# Autodesk Inventor assembly: Case inferiore completo
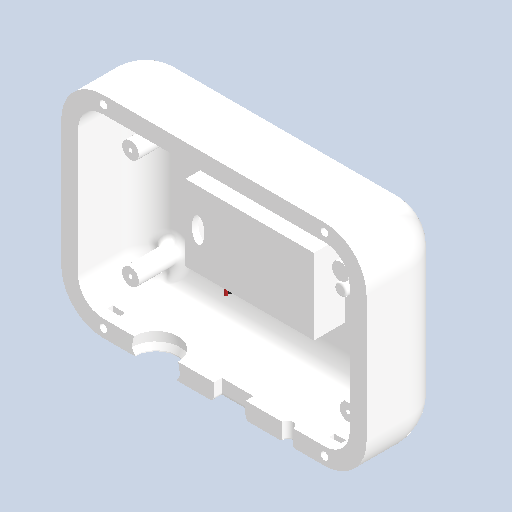
[picture p0: Inventor's stored thumbnail of the model, 512x512]
Saved by Autodesk Inventor 2023 (Build 270158000, 158)
## iProperties
Created: 2022-12-31
Part Number: Case inferiore completo
Document SubType Name: Assembly
Designer: Gabriele
Author: Gabriele
## Documents named in this file (3)
- C:\Users\Gabriele\Desktop\LAB\AY2223_I_Project-2\3D\Case\Case inferiore completo.iam
- C:\Users\Gabriele\Desktop\LAB\AY2223_I_Project-2\3D\Case\Case inferiore e batteria.iam
- C:\Users\Gabriele\Desktop\LAB\AY2223_I_Project-2\3D\Case\Coperchio.ipt
## Components (2 placed, 2 different names)
1. Case inferiore e batteria:1 [sub-assembly] — Inserimento:1
2. Coperchio:1 — Inserimento:1
## Relationships (1: Insert 1)
- Inserimento:1: Case inferiore e batteria:1 ↔ Coperchio:1
